# Autodesk Inventor assembly: holder+servo
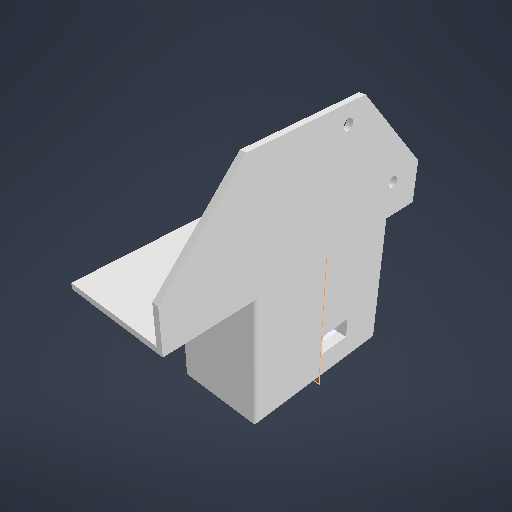
[picture p0: Inventor's stored thumbnail of the model, 512x512]
Saved by Autodesk Inventor 2026 (Build 300175050, 175E)
## iProperties
Created: 2025-05-22
Part Number: holder+servo
Document SubType Name: Assembly
Designer: sumit
Author: sumit
## Documents named in this file (4)
- C:\Users\sumit\Documents\GitHub\Robotics\Robotic-Arm\CAD\holder+servo.iam
- C:\Users\sumit\Documents\GitHub\Robotics\Robotic-Arm\CAD\servo_holder.ipt
- C:\Users\sumit\Documents\GitHub\Robotics\Robotic-Arm\CAD\Servo SC15.ipt
- C:\Users\sumit\Documents\GitHub\Robotics\Robotic-Arm\CAD\gripper servo mount.ipt
## Components (3 placed, 3 different names)
1. servo_holder:1 — Mate:1, Mate:2, Mate:3, Mate:4
2. Servo SC15:1 — Mate:1, Mate:2, Mate:3, Mate:5, Mate:6
3. gripper servo mount:1 — Mate:4, Mate:5, Mate:6
## Relationships (6: Mate 6)
- Mate:1: servo_holder:1 ↔ Servo SC15:1
- Mate:2: servo_holder:1 ↔ Servo SC15:1
- Mate:3: servo_holder:1 ↔ Servo SC15:1
- Mate:4: servo_holder:1 ↔ gripper servo mount:1
- Mate:5: Servo SC15:1 ↔ gripper servo mount:1
- Mate:6: Servo SC15:1 ↔ gripper servo mount:1
